# Autodesk Inventor assembly: ASM_Winch
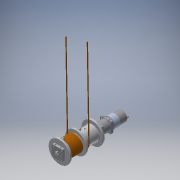
[picture p0: Inventor's stored thumbnail of the model, 180x180]
Saved by Autodesk Inventor 2016 (Build 200138000, 138)
## iProperties
Created: 2016-03-01
Part Number: ASM_Winch
Document SubType Name: Assembly
Designer: agmle
Mass: 583.203 g
Surface Area: 1073.75 cm^2
Volume: 434.881 cm^3
Density: 1.34106 g/cm^3
Author: agmle
## Documents named in this file (19)
- C:\Users\agmle\BitTorrent Sync\private\projects\Creekfleet_Timer\hardware\CAD\Remote\ASM_Winch.iam
- C:\Users\agmle\BitTorrent Sync\private\projects\Creekfleet_Timer\hardware\CAD\Remote\RS-550User Library-motor_rs-550-1.ipt
- C:\Users\agmle\BitTorrent Sync\private\projects\Creekfleet_Timer\hardware\CAD\Remote\P60_User Library-Banebots P60 16_1.ipt
- C:\Users\agmle\BitTorrent Sync\private\projects\Creekfleet_Timer\hardware\CAD\Remote\Drum.ipt
- C:\Users\agmle\Documents\Inventor\Content Center Files\R2016\en-US\GB 798-88\Eye bolt GB 798 M5 x 25.ipt
- C:\Users\agmle\BitTorrent Sync\private\projects\Creekfleet_Timer\hardware\CAD\Remote\Bearing_Block.ipt
- C:\Users\agmle\BitTorrent Sync\private\projects\Creekfleet_Timer\hardware\CAD\Remote\Drum_Key.ipt
- C:\Users\agmle\BitTorrent Sync\private\projects\Creekfleet_Timer\hardware\CAD\Remote\Drum_Axle.ipt
- C:\Users\agmle\Documents\Inventor\Content Center Files\R2016\en-US\BS 3673(3)\BS 3673_1 - S0050.ipt
- C:\Users\agmle\Documents\Inventor\Content Center Files\R2016\en-US\ANSI B18.3(08)\ANSI B18.3 - 10-24 UNC - 0.625(24).ipt
- C:\Users\agmle\Documents\Inventor\Content Center Files\R2016\en-US\IFI 512-S\IFI 512-S - 425.ipt
- C:\Users\agmle\BitTorrent Sync\private\projects\Creekfleet_Timer\hardware\CAD\Remote\Winding.ipt
- C:\Users\agmle\BitTorrent Sync\private\projects\Creekfleet_Timer\hardware\CAD\Remote\Unwinding.ipt
- C:\Users\agmle\BitTorrent Sync\private\projects\Creekfleet_Timer\hardware\CAD\Remote\ASM_Winch\AIP\FEA\br0snzahs.fins
- C:\Users\agmle\BitTorrent Sync\private\projects\Creekfleet_Timer\hardware\CAD\Remote\ASM_Winch\AIP\FEA\br0snzahs.fsat
- C:\Users\agmle\BitTorrent Sync\private\projects\Creekfleet_Timer\hardware\CAD\Remote\ASM_Winch\AIP\FEA\br0snzahs.ftes
- C:\Users\agmle\BitTorrent Sync\private\projects\Creekfleet_Timer\hardware\CAD\Remote\ASM_Winch\AIP\FEA\br0snzahs.fwiz
- C:\Users\agmle\BitTorrent Sync\private\projects\Creekfleet_Timer\hardware\CAD\Remote\ASM_Winch\AIP\FEA\br0te62ps.fmsh
- C:\Users\agmle\BitTorrent Sync\private\projects\Creekfleet_Timer\hardware\CAD\Remote\ASM_Winch\AIP\FEA\br0te62pt.fres
## Components (14 placed, 12 different names)
1. RS-550User Library-motor_rs-550-1:1 — Mate:3, Mate:4
2. P60_User Library-Banebots P60 16_1:1 — Mate:1, Flush:1, Mate:2, Mate:3, Mate:4, Flush:2, Mate:17, Mate:18
3. Drum:1 — Mate:1, Flush:1, Mate:2, Insert:1, Insert:2, Mate:5, Mate:6, Flush:3, Mate:8, Mate:9, Insert:4, Mate:11, Mate:12, Mate:15, Mate:16
4. Bolt GB/T 798-1988 M5 x 25:1 — Insert:1, Flush:4, Angle:2, Tangent:1
5. Bolt GB/T 798-1988 M5 x 25:2 — Insert:2, Flush:4, Angle:1, Tangent:2
6. Bearing_Block:1 — Mate:5, Mate:6, Flush:2
7. Drum_Key:1 — Flush:3, Mate:8, Mate:9, Mate:10, Mate:13, Mate:14
8. Drum_Axle:1 — Insert:3, Mate:10, Insert:5
9. BS 3673 : Part 1 - Inch S0050:1 — Insert:3, Insert:4
10. Hexagon Socket Set Screw - Flat Point - Inch 10-24 UNC x 0.625:2 — Mate:11, Mate:13
11. Hexagon Socket Set Screw - Flat Point - Inch 10-24 UNC x 0.625:1 — Mate:12, Mate:14
12. Pin - Slotted Spring (Metric) (IFI) 4:1 — Insert:5
13. Winding:1 — Mate:15, Angle:1, Tangent:2
14. Unwinding:1 — Mate:16, Angle:2, Tangent:1
## Relationships (30: Mate 17, Insert 5, Flush 4, Angle 2, Tangent 2)
- Mate:1: P60_User Library-Banebots P60 16_1:1 ↔ Drum:1
- Flush:1: P60_User Library-Banebots P60 16_1:1 ↔ Drum:1
- Mate:2: P60_User Library-Banebots P60 16_1:1 ↔ Drum:1
- Mate:3: RS-550User Library-motor_rs-550-1:1 ↔ P60_User Library-Banebots P60 16_1:1
- Mate:4: RS-550User Library-motor_rs-550-1:1 ↔ P60_User Library-Banebots P60 16_1:1
- Insert:1: Drum:1 ↔ Bolt GB/T 798-1988 M5 x 25:1
- Insert:2: Drum:1 ↔ Bolt GB/T 798-1988 M5 x 25:2
- Mate:5: Drum:1 ↔ Bearing_Block:1
- Mate:6: Drum:1 ↔ Bearing_Block:1
- Flush:2: P60_User Library-Banebots P60 16_1:1 ↔ Bearing_Block:1
- Flush:3: Drum:1 ↔ Drum_Key:1
- Mate:8: Drum:1 ↔ Drum_Key:1
- Mate:9: Drum:1 ↔ Drum_Key:1
- Insert:3: Drum_Axle:1 ↔ BS 3673 : Part 1 - Inch S0050:1
- Mate:10: Drum_Key:1 ↔ Drum_Axle:1
- Insert:4: Drum:1 ↔ BS 3673 : Part 1 - Inch S0050:1
- Mate:11: Drum:1 ↔ Hexagon Socket Set Screw - Flat Point - Inch 10-24 UNC x 0.625:2
- Mate:12: Drum:1 ↔ Hexagon Socket Set Screw - Flat Point - Inch 10-24 UNC x 0.625:1
- Mate:13: Drum_Key:1 ↔ Hexagon Socket Set Screw - Flat Point - Inch 10-24 UNC x 0.625:2
- Mate:14: Drum_Key:1 ↔ Hexagon Socket Set Screw - Flat Point - Inch 10-24 UNC x 0.625:1
- Insert:5: Drum_Axle:1 ↔ Pin - Slotted Spring (Metric) (IFI) 4:1
- Flush:4: Bolt GB/T 798-1988 M5 x 25:1 ↔ Bolt GB/T 798-1988 M5 x 25:2
- Mate:15: Drum:1 ↔ Winding:1
- Angle:1 (179 deg): Bolt GB/T 798-1988 M5 x 25:2 ↔ Winding:1
- Mate:16: Drum:1 ↔ Unwinding:1
- Angle:2 (179 deg): Bolt GB/T 798-1988 M5 x 25:1 ↔ Unwinding:1
- Mate:17: P60_User Library-Banebots P60 16_1:1
- Mate:18: P60_User Library-Banebots P60 16_1:1
- Tangent:1: Bolt GB/T 798-1988 M5 x 25:1 ↔ Unwinding:1
- Tangent:2: Bolt GB/T 798-1988 M5 x 25:2 ↔ Winding:1
## Named parameters: sa_1 = 980.999, sa_0 = 3389.54, sa_2 = 564.924
note: some values were not read from the file. Shown as the stored number, unit unknown: "sa_1", "sa_0", "sa_2".
